# Autodesk Inventor assembly: Module Cradle V1
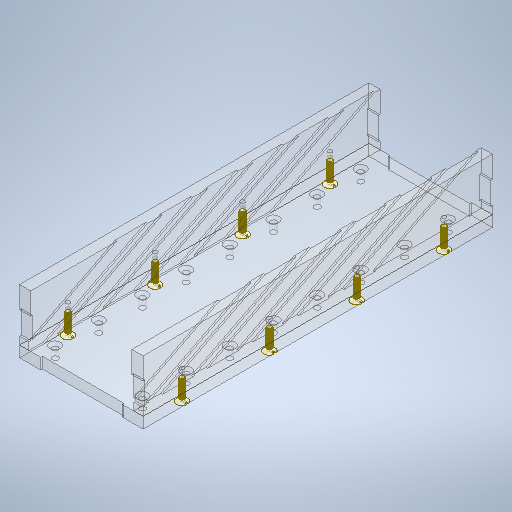
[picture p0: Inventor's stored thumbnail of the model, 512x512]
Saved by Autodesk Inventor 2025 (Build 290162000, 162)
## iProperties
Created: 2024-03-20
Part Number: Module Cradle V1
Document SubType Name: Assembly
Designer: cfang
Author: cfang
## Documents named in this file (5)
- C:\Users\cfang\Desktop\nebraska-silicon-lab\Hardware\ETL\Irradiation Fixture\Module Cradle V1.iam
- C:\Users\cfang\Desktop\nebraska-silicon-lab\Hardware\ETL\Irradiation Fixture\Module Cradle Left V1.ipt
- C:\Users\cfang\Desktop\nebraska-silicon-lab\Hardware\ETL\Irradiation Fixture\Module Cradle Base V1.ipt
- C:\Users\cfang\Desktop\nebraska-silicon-lab\Hardware\ETL\Irradiation Fixture\Module Cradle Right V1.ipt
- C:\Users\cfang\Desktop\nebraska-silicon-lab\Hardware\ETL\Irradiation Fixture\93840A122_Off-White Nylon Slotted Flat Head Screws\93840A122_Off-White Nylon Slotted Flat Head Screws.ipt
## Components (11 placed, 4 different names)
1. Module Cradle Left V1:2 — Mate:1, Flush:2, Flush:5
2. Module Cradle Base V1:1 — Mate:1, Flush:2, Mate:2, Flush:3, Flush:4, Flush:5, Insert:1, Insert:2, Insert:3, Insert:4, Insert:5, Insert:6, Insert:7, Insert:8
3. Module Cradle Right V1:1 — Mate:2, Flush:3, Flush:4
4. 93840A122_Off-White Nylon Slotted Flat Head Screws:1 — Insert:1
5. 93840A122_Off-White Nylon Slotted Flat Head Screws:2 — Insert:3
6. 93840A122_Off-White Nylon Slotted Flat Head Screws:3 — Insert:7
7. 93840A122_Off-White Nylon Slotted Flat Head Screws:4 — Insert:2
8. 93840A122_Off-White Nylon Slotted Flat Head Screws:5 — Insert:4
9. 93840A122_Off-White Nylon Slotted Flat Head Screws:6 — Insert:8
10. 93840A122_Off-White Nylon Slotted Flat Head Screws:7 — Insert:6
11. 93840A122_Off-White Nylon Slotted Flat Head Screws:8 — Insert:5
## Relationships (14: Insert 8, Flush 4, Mate 2)
- Mate:1: Module Cradle Left V1:2 ↔ Module Cradle Base V1:1
- Flush:2: Module Cradle Left V1:2 ↔ Module Cradle Base V1:1
- Mate:2: Module Cradle Base V1:1 ↔ Module Cradle Right V1:1
- Flush:3: Module Cradle Base V1:1 ↔ Module Cradle Right V1:1
- Flush:4: Module Cradle Base V1:1 ↔ Module Cradle Right V1:1
- Flush:5: Module Cradle Left V1:2 ↔ Module Cradle Base V1:1
- Insert:1: Module Cradle Base V1:1 ↔ 93840A122_Off-White Nylon Slotted Flat Head Screws:1
- Insert:2: Module Cradle Base V1:1 ↔ 93840A122_Off-White Nylon Slotted Flat Head Screws:4
- Insert:3: Module Cradle Base V1:1 ↔ 93840A122_Off-White Nylon Slotted Flat Head Screws:2
- Insert:4: Module Cradle Base V1:1 ↔ 93840A122_Off-White Nylon Slotted Flat Head Screws:5
- Insert:5: Module Cradle Base V1:1 ↔ 93840A122_Off-White Nylon Slotted Flat Head Screws:8
- Insert:6: Module Cradle Base V1:1 ↔ 93840A122_Off-White Nylon Slotted Flat Head Screws:7
- Insert:7: Module Cradle Base V1:1 ↔ 93840A122_Off-White Nylon Slotted Flat Head Screws:3
- Insert:8: Module Cradle Base V1:1 ↔ 93840A122_Off-White Nylon Slotted Flat Head Screws:6
